# Autodesk Inventor assembly: gyroPhone07
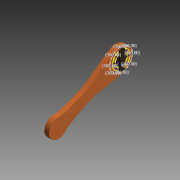
[picture p0: Inventor's stored thumbnail of the model, 180x180]
Saved by Autodesk Inventor 2013 (Build 170138000, 138)
## iProperties
Created: 2013-01-21
Part Number: gyroPhone07
Document SubType Name: Assembly
Designer: Nano
Author: Nano
## Documents named in this file (5)
- C:\Users\Nano\Documents\InventorByron\InventorMasterProject\gyroPhone01\gyroPhone07.iam
- C:\Users\Nano\Documents\InventorByron\InventorMasterProject\gyroPhone01\wheelAssembly01.iam
- C:\Users\Nano\Documents\InventorByron\InventorMasterProject\gyroPhone01\motorDriveWheelAssembly.iam
- C:\Users\Nano\Documents\InventorByron\InventorMasterProject\gyroPhone01\body_11.ipt
- C:\Users\Nano\Documents\InventorByron\InventorMasterProject\gyroPhone01\pivotMech01.ipt
## Components (4 placed, 4 different names)
1. wheelAssembly01:1 [sub-assembly] — Mate:1, Mate:2, Flush:1, Flush:2, Flush:3, Flush:4
2. motorDriveWheelAssembly:1 [sub-assembly] — Mate:1, Mate:2
3. body_11:1 — Flush:1, Flush:2
4. pivotMech01:1 — Flush:3, Flush:4
## Relationships (6: Flush 4, Mate 2)
- Mate:1 (3.175 mm): wheelAssembly01:1 ↔ motorDriveWheelAssembly:1
- Mate:2: wheelAssembly01:1 ↔ motorDriveWheelAssembly:1
- Flush:1: wheelAssembly01:1 ↔ body_11:1
- Flush:2: wheelAssembly01:1 ↔ body_11:1
- Flush:3: wheelAssembly01:1 ↔ pivotMech01:1
- Flush:4 (3.175 mm): wheelAssembly01:1 ↔ pivotMech01:1
